# Autodesk Inventor assembly: oktagon
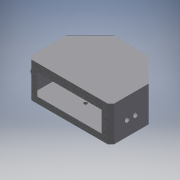
[picture p0: Inventor's stored thumbnail of the model, 180x180]
Saved by Autodesk Inventor 2018.2 (Build 222227000, 227)
## iProperties
Created: 2018-08-16
Part Number: oktagon
Material: Generisch
Document SubType Name: Assembly
Designer: PRYADUN
Author: PRYADUN
## Documents named in this file (3)
- U:\COSIMA-Laserstar\CAD\oktagon.iam
- U:\COSIMA-Laserstar\CAD\oktagonOben_v2.ipt
- U:\COSIMA-Laserstar\CAD\oktagonUnten_v2.ipt
## Components (2 placed, 2 different names)
1. oktagonOben_v2:1 — Passend:1, Fluchtend:1, Fluchtend:2
2. oktagonUnten_v2:1 — Passend:1, Fluchtend:1, Fluchtend:2
## Relationships (3: Flush 2, Mate 1)
- Passend:1 [Mate]: oktagonOben_v2:1 ↔ oktagonUnten_v2:1
- Fluchtend:1 [Flush]: oktagonOben_v2:1 ↔ oktagonUnten_v2:1
- Fluchtend:2 [Flush]: oktagonOben_v2:1 ↔ oktagonUnten_v2:1
